# Autodesk Inventor assembly: Modificacion_altura
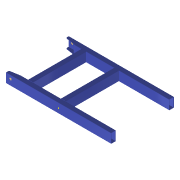
[picture p0: Inventor's stored thumbnail of the model, 180x180]
Saved by Autodesk Inventor 2020 (Build 240168000, 168)
## iProperties
Created: 2020-02-24
Part Number: Modificacion_altura
Document SubType Name: Assembly
Designer: Juan Carlos Botero
Author: Juan Carlos Botero
## Documents named in this file (6)
- D:\Drives\OneDrive\Carlos_2\02 TRABAJOS\MULTIPLO\Conveyor\ENSAMBLE - Copy\Modificacion_altura.iam
- D:\Drives\OneDrive\Carlos_2\02 TRABAJOS\MULTIPLO\Conveyor\ENSAMBLE - Copy\Perfil_banda-02.ipt
- D:\Drives\OneDrive\Carlos_2\02 TRABAJOS\MULTIPLO\Conveyor\ENSAMBLE\Arandela pivote.ipt
- D:\Drives\OneDrive\Carlos_2\02 TRABAJOS\MULTIPLO\Conveyor\ENSAMBLE - Copy\Perfil_banda-02_MIR.ipt
- D:\Drives\OneDrive\Carlos_2\02 TRABAJOS\MULTIPLO\Conveyor\ENSAMBLE - Copy\Refuerzo_modificacion.ipt
- D:\Drives\OneDrive\Carlos_2\02 TRABAJOS\MULTIPLO\Conveyor\ENSAMBLE\Buje.ipt
## Components (8 placed, 5 different names)
1. Perfil_banda-02:1 — Flush:5, Flush:7, Flush:9
2. Arandela pivote:1 — Mate:8, Flush:3, Flush:4
3. Perfil_banda-02_MIR:1 — Mate:9, Angle:1, Flush:5, Mate:11, Flush:6, Mate:12, Flush:10
4. Refuerzo_modificacion:1 — Mate:11, Flush:6, Flush:10
5. Refuerzo_modificacion:2 — Flush:7, Flush:9
6. Buje:1 — Mate:10, Flush:8
7. Buje:2 — Mate:8, Flush:3
8. Arandela pivote:2 — Mate:9, Mate:10, Angle:1, Flush:4, Mate:12, Flush:8
## Relationships (19: Mate 9, Flush 9, Angle 1)
- [Mate]: Perfil_banda-02:1 ↔ Arandela pivote:1
- [Mate]: Perfil_banda-02:1 ↔ Arandela pivote:1
- [Mate]: Perfil_banda-02:1 ↔ Refuerzo_modificacion:1
- [Mate]: Perfil_banda-02:1 ↔ Refuerzo_modificacion:2
- [Flush]: Refuerzo_modificacion:1 ↔ Refuerzo_modificacion:2
- Mate:8: Arandela pivote:1 ↔ Buje:2
- Flush:3: Arandela pivote:1 ↔ Buje:2
- Mate:9: Perfil_banda-02_MIR:1 ↔ Arandela pivote:2
- Mate:10: Buje:1 ↔ Arandela pivote:2
- Angle:1 (0 deg): Perfil_banda-02_MIR:1 ↔ Arandela pivote:2
- Flush:4: Arandela pivote:1 ↔ Arandela pivote:2
- Flush:5: Perfil_banda-02:1 ↔ Perfil_banda-02_MIR:1
- Mate:11: Perfil_banda-02_MIR:1 ↔ Refuerzo_modificacion:1
- Flush:6: Perfil_banda-02_MIR:1 ↔ Refuerzo_modificacion:1
- Flush:7: Perfil_banda-02:1 ↔ Refuerzo_modificacion:2
- Mate:12: Perfil_banda-02_MIR:1 ↔ Arandela pivote:2
- Flush:8: Buje:1 ↔ Arandela pivote:2
- Flush:9 (180 mm): Perfil_banda-02:1 ↔ Refuerzo_modificacion:2
- Flush:10 (537 mm): Perfil_banda-02_MIR:1 ↔ Refuerzo_modificacion:1
